# Autodesk Inventor assembly: IndexL1
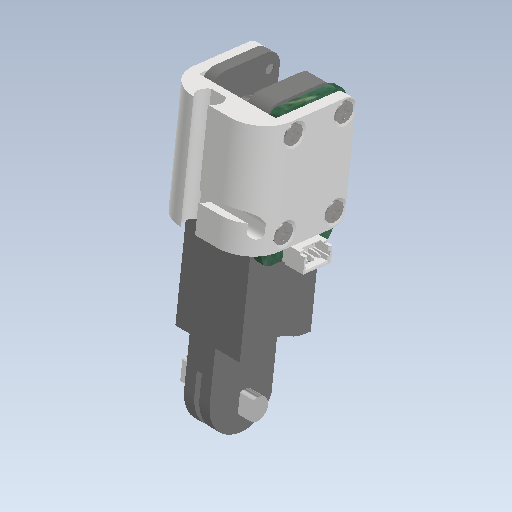
[picture p0: Inventor's stored thumbnail of the model, 512x512]
Saved by Autodesk Inventor 2020 (Build 240168000, 168)
## iProperties
Created: 2020-04-30
Part Number: IndexL1
Document SubType Name: Assembly
Designer: sami_
Author: sami_
## Documents named in this file (10)
- C:\Users\sami_\Documents\V1.6\IndexL1.iam
- C:\Users\sami_\Documents\V1.6\Workgroups\NotInProject\INDEX\L1Index.ipt
- C:\Users\sami_\Documents\V1.6\Libraries\Content Center Files\en-US\ISO 1224-1 M\ISO 1224-1 - 17 - 4 x 7 x 2.ipt
- C:\Users\sami_\Documents\V1.6\Workgroups\NotInProject\INDEX\PotentiometerAssembly.iam
- C:\Users\sami_\Documents\V1.6\Libraries\Content Center Files\en-US\ISO 7089\ISO 7089 - 1.6 - 140 HV(1).ipt
- C:\Users\sami_\Documents\V1.6\Workgroups\NotInProject\SHAFT.ipt
- C:\Users\sami_\Documents\V1.6\Workgroups\NotInProject\fingerpanel_MIR.ipt
- C:\Users\sami_\Documents\V1.6\Libraries\Content Center Files\en-US\AS 1427(04)\AS 1427 - M2 x 8(5) I.ipt
- C:\Users\sami_\Documents\V1.6\Libraries\Content Center Files\en-US\AS 1427(04)\AS 1427 - M2 x 4(5) I.ipt
- C:\Users\sami_\Documents\V1.6\Libraries\Content Center Files\en-US\ISO 7089\ISO 7089 - 4 - 140 HV(1).ipt
## Components (24 placed, 9 different names)
1. L1Index:1
2. ISO 1224-1 (Metric) 17 - 4 x 7 x 2:1
3. ISO 7089 4:2
4. ISO 7089 4:1
5. ISO 1224-1 (Metric) 17 - 4 x 7 x 2:2
6. PotentiometerAssembly:1 [sub-assembly]
7. ISO 7089 1.6:1
8. ISO 7089 1.6:2
9. ISO 7089 1.6:3
10. ISO 7089 1.6:4
11. ISO 7089 1.6:5
12. ISO 7089 1.6:6
13. ISO 7089 1.6:7
14. SHAFT:2
15. ISO 7089 1.6:8
16. fingerpanel_MIR:1
17. AS 1427 H - Metric M2 x 8:1
18. AS 1427 H - Metric M2 x 8:2
19. AS 1427 H - Metric M2 x 8:3
20. AS 1427 H - Metric M2 x 8:4
21. AS 1427 H - Metric M2 x 4:1
22. AS 1427 H - Metric M2 x 4:2
23. AS 1427 H - Metric M2 x 4:3
24. AS 1427 H - Metric M2 x 4:4
## Relationships (24: Mate 10, Insert 8, WeldJoint 6)
- [WeldJoint]: L1Index:1 ↔ ISO 1224-1 (Metric) 17 - 4 x 7 x 2:1
- [WeldJoint]: L1Index:1 ↔ ISO 1224-1 (Metric) 17 - 4 x 7 x 2:2
- [WeldJoint] (-0.6 mm): L1Index:1 ↔ PotentiometerAssembly:1
- [Insert]: L1Index:1 ↔ ISO 7089 1.6:1
- [Insert]: L1Index:1 ↔ ISO 7089 1.6:2
- [Insert]: L1Index:1 ↔ ISO 7089 1.6:3
- [Insert]: L1Index:1 ↔ ISO 7089 1.6:4
- [Insert]: ISO 7089 1.6:4 ↔ ISO 7089 1.6:5
- [Insert]: ISO 7089 1.6:3 ↔ ISO 7089 1.6:6
- [Insert]: ISO 7089 1.6:2 ↔ ISO 7089 1.6:7
- [Insert]: ISO 7089 1.6:1 ↔ ISO 7089 1.6:8
- [WeldJoint]: PotentiometerAssembly:1 ↔ fingerpanel_MIR:1
- [Mate]: fingerpanel_MIR:1 ↔ AS 1427 H - Metric M2 x 8:1
- [Mate]: fingerpanel_MIR:1 ↔ AS 1427 H - Metric M2 x 8:2
- [Mate]: fingerpanel_MIR:1 ↔ AS 1427 H - Metric M2 x 8:3
- [Mate]: fingerpanel_MIR:1 ↔ AS 1427 H - Metric M2 x 8:4
- [Mate]: fingerpanel_MIR:1 ↔ AS 1427 H - Metric M2 x 4:1
- [Mate]: fingerpanel_MIR:1 ↔ AS 1427 H - Metric M2 x 4:2
- [Mate]: fingerpanel_MIR:1 ↔ AS 1427 H - Metric M2 x 4:3
- [Mate]: fingerpanel_MIR:1 ↔ AS 1427 H - Metric M2 x 4:4
- [Mate]: L1Index:1 ↔ SHAFT:2
- [Mate]: L1Index:1 ↔ SHAFT:2
- [WeldJoint]: ISO 1224-1 (Metric) 17 - 4 x 7 x 2:1 ↔ ISO 7089 4:1
- [WeldJoint]: L1Index:1 ↔ ISO 7089 4:2
